# Autodesk Inventor assembly: Spike H
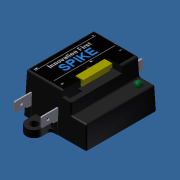
[picture p0: Inventor's stored thumbnail of the model, 180x180]
Saved by Autodesk Inventor 2012 (Build 160160000, 160)
## iProperties
Shininess: 64.0
Length Units: 11270
Angle Units: 11279
Time Units: 11290
Mass Units: 11283
Length Display Precision: 3
Angle Display Precision: 2
Compacted: True
Created: 2006-01-06
Part Number: Spike H
Document SubType Name: Assembly
Designer: Owner
Mass: 25.5355 g
Surface Area: 243.741 cm^2
Volume: 18.4281 cm^3
Density: 1.38569 g/cm^3
Density: 0.0
Volumn: 0.0
Area: 0.0
PropertySet Name: Model Information
Control State: 0
Master: False
Checked Out: False
Author: Owner
## Documents named in this file (9)
- C:\Users\Edward\Documents\masters\CAD\Spike\Spike H.iam
- C:\Users\Edward\Documents\masters\CAD\Spike\Spike Bottom Cover.ipt
- C:\Users\Edward\Documents\masters\CAD\Spike\Spike PCB.ipt
- C:\Users\Edward\Documents\masters\CAD\Spike\Spike Female Terminal.ipt
- C:\Users\Edward\Documents\masters\CAD\Spike\1x3 Header Connector.ipt
- C:\Users\Edward\Documents\masters\CAD\Spike\Spike Male Terminal.ipt
- C:\Users\Edward\Documents\masters\CAD\Spike\ATO Fuse.ipt
- C:\Users\Edward\Documents\masters\CAD\Spike\Spike Top Cover.ipt
- C:\Users\Edward\Documents\masters\CAD\Spike\LED - Green.ipt
## Components (12 placed, 8 different names)
1. Spike Bottom Cover:1 — Mate:1, Mate:2, Mate:3, Mate:11, Mate:12, Flush:9
2. Spike PCB:1 — Mate:1, Mate:2, Mate:3, Mate:4, Flush:1, Mate:5, Mate:6, Flush:2, Flush:3, Mate:7, Flush:4, Flush:5, Mate:8, Flush:6, Flush:7, Flush:8
3. 1x3 Header Connector:1 — Mate:6, Flush:2, Flush:3
4. ATO Fuse:1 — Mate:9, Mate:10, Flush:8
5. Spike Top Cover:1 — Mate:11, Mate:12, Flush:9, Mate:13, Mate:14
6. LED - Green:1 — Mate:13, Mate:14
7. Spike Female Terminal:1 — Mate:4, Flush:1, Mate:5, Mate:9, Mate:10
8. Spike Female Terminal:2
9. Spike Male Terminal:2 — Mate:8, Flush:6, Flush:7
10. Spike Male Terminal:1 — Mate:7, Flush:4, Flush:5
11. Spike Male Terminal:3
12. Spike Male Terminal:4
## Component patterns: (2 elements, first: Spike Female Terminal:1), (2 elements, first: Spike Male Terminal:2 + Spike Male Terminal:1)
## Relationships (23: Mate 14, Flush 9)
- Mate:1: Spike Bottom Cover:1 ↔ Spike PCB:1
- Mate:2: Spike Bottom Cover:1 ↔ Spike PCB:1
- Mate:3: Spike Bottom Cover:1 ↔ Spike PCB:1
- Mate:4 (0.1 mm): Spike PCB:1 ↔ Spike Female Terminal:1
- Flush:1 (-14.8 mm): Spike PCB:1 ↔ Spike Female Terminal:1
- Mate:5 (-14.18 mm): Spike PCB:1 ↔ Spike Female Terminal:1
- Mate:6: Spike PCB:1 ↔ 1x3 Header Connector:1
- Flush:2 (11.65 mm): Spike PCB:1 ↔ 1x3 Header Connector:1
- Flush:3 (1 mm): Spike PCB:1 ↔ 1x3 Header Connector:1
- Mate:7 (0.1 mm): Spike PCB:1 ↔ Spike Male Terminal:1
- Flush:4 (0.5 mm): Spike PCB:1 ↔ Spike Male Terminal:1
- Flush:5 (1.75 mm): Spike PCB:1 ↔ Spike Male Terminal:1
- Mate:8: Spike PCB:1 ↔ Spike Male Terminal:2
- Flush:6 (0.5 mm): Spike PCB:1 ↔ Spike Male Terminal:2
- Flush:7 (1.75 mm): Spike PCB:1 ↔ Spike Male Terminal:2
- Mate:9: ATO Fuse:1 ↔ Spike Female Terminal:1
- Mate:10 (1 mm): ATO Fuse:1 ↔ Spike Female Terminal:1
- Flush:8 (13.8 mm): Spike PCB:1 ↔ ATO Fuse:1
- Mate:11: Spike Bottom Cover:1 ↔ Spike Top Cover:1
- Mate:12: Spike Bottom Cover:1 ↔ Spike Top Cover:1
- Flush:9: Spike Bottom Cover:1 ↔ Spike Top Cover:1
- Mate:13: Spike Top Cover:1 ↔ LED - Green:1
- Mate:14 (-6.5 mm): Spike Top Cover:1 ↔ LED - Green:1
